# Autodesk Inventor assembly: Leg_joint_roll_pitch
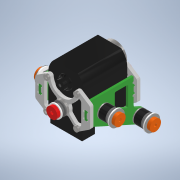
[picture p0: Inventor's stored thumbnail of the model, 180x180]
Saved by Autodesk Inventor 2020.4 (Build 244396000, 396)
## iProperties
Part Number: Leg_joint_roll_pitch
Document SubType Name: Assembly
Designer: Masato Kubotera
Mass: 101.309 g
Surface Area: 368.925 cm^2
Volume: 74.117 cm^3
Density: 1.36688 g/cm^3
Author: Masato Kubotera
## Documents named in this file (22)
- C:\Users\Masato\Documents\Inventor\CIT Brains_Inventor\SUSTAINA-OP\LowerBody\Leg_joit\Leg_joint_roll_pitch.iam
- C:\Users\Masato\Documents\Inventor\CIT Brains_Inventor\SUSTAINA-OP\LowerBody\Leg_joit\Leg_joint_pitch_frame.ipt
- C:\Users\Masato\Documents\Inventor\CIT Brains_Inventor\SUSTAINA-OP\LowerBody\Leg_joit\Leg_joint_roll_frame.ipt
- C:\Users\Masato\Documents\Inventor\CIT Brains_Inventor\SUSTAINA-OP\ReadyMade\KONDO\B3M-SC-1170-A.ipt
- C:\Users\Masato\Documents\Inventor\CIT Brains_Inventor\SUSTAINA-OP\ReadyMade\Screw\M2_6-20.ipt
- C:\Users\Masato\Documents\Inventor\CIT Brains_Inventor\SUSTAINA-OP\ReadyMade\Screw\M2_6-15.ipt
- C:\Users\Masato\Documents\Inventor\CIT Brains_Inventor\SUSTAINA-OP\ReadyMade\Bush\80F-0603.ipt
- C:\Users\Masato\Documents\Inventor\CIT Brains_Inventor\SUSTAINA-OP\ReadyMade\Washer\CC-0612-50B.ipt
- C:\Users\Masato\Documents\Inventor\CIT Brains_Inventor\SUSTAINA-OP\ReadyMade\InsertNut\SF419.ipt
- C:\Users\Masato\Documents\Inventor\CIT Brains_Inventor\SUSTAINA-OP\ReadyMade\Washer\UUW-0412-10H.ipt
- C:\Users\Masato\Documents\Inventor\CIT Brains_Inventor\SUSTAINA-OP\ReadyMade\Spacer\SLSBF6-39.5-M4-N4.ipt
- C:\Users\Masato\Documents\Inventor\CIT Brains_Inventor\SUSTAINA-OP\ReadyMade\Screw\DBTS4-11-6-DHC.ipt
- C:\Users\Masato\Documents\Inventor\CIT Brains_Inventor\SUSTAINA-OP\ReadyMade\Screw\DBTS4-5-5-DHC.ipt
- C:\Users\Masato\Documents\Inventor\CIT Brains_Inventor\SUSTAINA-OP\ReadyMade\Screw\DBTS4-10-4-DHC.ipt
- C:\Users\Masato\Documents\Inventor\CIT Brains_Inventor\SUSTAINA-OP\ReadyMade\InsertNut\S4-05-3W.ipt
- C:\Users\Masato\Documents\Inventor\CIT Brains_Inventor\SUSTAINA-OP\ReadyMade\KONDO\ClampHorn.ipt
- C:\Users\Masato\Documents\Inventor\CIT Brains_Inventor\SUSTAINA-OP\ReadyMade\Screw\620103008.ipt
- C:\Users\Masato\Documents\Inventor\CIT Brains_Inventor\SUSTAINA-OP\ReadyMade\Screw\DBTS4-11-8-DHC.ipt
- C:\Users\Masato\Documents\Inventor\CIT Brains_Inventor\SUSTAINA-OP\ReadyMade\Washer\UUW-0614-05H.ipt
- C:\Users\Masato\Documents\Inventor\CIT Brains_Inventor\SUSTAINA-OP\ReadyMade\Washer\TT-0612-10.ipt
- C:\Users\Masato\Documents\Inventor\CIT Brains_Inventor\SUSTAINA-OP\ReadyMade\Washer\TT-0814-10.ipt
- C:\Users\Masato\Documents\Inventor\CIT Brains_Inventor\SUSTAINA-OP\ReadyMade\Washer\CCC-0612-65B.ipt
## Components (52 placed, 21 different names)
1. B3M-SC-1170-A:1 — 挿入:1, 挿入:2, 挿入:3, 挿入:4, 挿入:11, 挿入:12, 挿入:13, 挿入:14, メイト:1, メイト:2, フラッシュ:1, 挿入:49, 角度:3, 挿入:50
2. Leg_joint_roll_frame:1 — 挿入:1, 挿入:2, 挿入:3, 挿入:4, 挿入:5, 挿入:6, 挿入:7, 挿入:8, 挿入:9, 挿入:10, 角度:1, フラッシュ:2, メイト:3, メイト:4, メイト:5
3. Leg_joint_roll_frame:2 — 挿入:11, 挿入:12, 挿入:13, 挿入:14, 挿入:15, 挿入:16, 挿入:17, 挿入:18, 角度:2, 角度:4
4. Leg_joint_pitch_frame:1 — フラッシュ:3, 挿入:19, フラッシュ:4, メイト:5, 挿入:20, 挿入:21, 挿入:22
5. Leg_joint_pitch_frame:2 — フラッシュ:2, フラッシュ:3, フラッシュ:4, メイト:3, メイト:4, 挿入:23, 挿入:24, 挿入:25, 挿入:26
6. 80F-0603:1 — 挿入:43
7. 80F-0603:2 — 挿入:44
8. 80F-0603:3 — 挿入:243
9. 80F-0603:4 — 挿入:242
10. 80F-0603:5 — 挿入:244
11. 80F-0603:6 — 挿入:245
12. UUW-0412-10BH:1 — 挿入:9, 挿入:27
13. UUW-0412-10BH:2 — 挿入:17, 挿入:28, 挿入:33
14. UUW-0412-10BH:3 — 挿入:19, 挿入:226, 挿入:241
15. UUW-0412-10BH:4 — 挿入:22, 挿入:35, 挿入:240
16. UUW-0412-10BH:5 — 挿入:23, 挿入:227, 挿入:239
17. UUW-0412-10BH:6 — 挿入:26, 挿入:37, 挿入:238
18. UUW-0412-10BH:7 — 挿入:27, 挿入:38, 挿入:43
19. CC-0612-50B:5 — 挿入:28, 挿入:44
20. SF419:1 — 挿入:25
21. SF419:2 — 挿入:20
22. S4-05-3W:1 — 挿入:10, 角度:1
23. S4-05-3W:2 — 挿入:18, 角度:2
24. SLSBF6-39.5-M4-N4:1 — 挿入:21, 挿入:24, 角度:4
25. DBS4-5-5:1 — 挿入:38, 挿入:232
26. DBTS4-11-6:3 — 挿入:37, 挿入:229
27. DBTS4-11-6:4 — 挿入:35, 挿入:230
28. DBTS4-10-4:1 — 挿入:33, 挿入:233
29. ClampHorn:1 — 挿入:49, 角度:3
30. 620103008:1 — 挿入:50
31. DBTS4-11-8:1 — 挿入:226, 挿入:231
32. DBTS4-11-8:2 — 挿入:227, 挿入:228
33. UUW-0614-05BH:1 — 挿入:228, 挿入:234
34. UUW-0614-05BH:2 — 挿入:229, 挿入:235
35. UUW-0614-05BH:3 — 挿入:230, 挿入:236
36. UUW-0614-05BH:4 — 挿入:231, 挿入:237
37. TT-0612-10:1 — 挿入:233
38. TT-0612-10:2 — 挿入:232
39. TT-0814-10:1 — 挿入:234
40. TT-0814-10:2 — 挿入:235
41. TT-0814-10:3 — 挿入:237
42. TT-0814-10:4 — 挿入:236
43. CCC-0612-65B:1 — 挿入:238, 挿入:245
44. CCC-0612-65B:2 — 挿入:241, 挿入:243
45. CCC-0612-65B:3 — 挿入:239, 挿入:244
46. CCC-0612-65B:4 — 挿入:240, 挿入:242
47. M2_6-20:1 — 挿入:7
48. M2_6-20:2 — 挿入:8
49. M2_6-20:3 — 挿入:5
50. M2_6-20:4 — 挿入:6
51. M2_6-15:2 — 挿入:16
52. M2_6-15:3 — 挿入:15
## Relationships (69: Insert 56, Mate 5, Flush 4, Angle 4)
- フラッシュ:1 [Flush]: B3M-SC-1170-A:1
- メイト:1 [Mate]: B3M-SC-1170-A:1
- メイト:2 [Mate]: B3M-SC-1170-A:1
- 挿入:1 [Insert]: B3M-SC-1170-A:1 ↔ Leg_joint_roll_frame:1
- 挿入:2 [Insert]: B3M-SC-1170-A:1 ↔ Leg_joint_roll_frame:1
- 挿入:3 [Insert]: B3M-SC-1170-A:1 ↔ Leg_joint_roll_frame:1
- 挿入:4 [Insert]: B3M-SC-1170-A:1 ↔ Leg_joint_roll_frame:1
- 挿入:5 [Insert]: Leg_joint_roll_frame:1 ↔ M2_6-20:3
- 挿入:6 [Insert]: Leg_joint_roll_frame:1 ↔ M2_6-20:4
- 挿入:7 [Insert]: Leg_joint_roll_frame:1 ↔ M2_6-20:1
- 挿入:8 [Insert]: Leg_joint_roll_frame:1 ↔ M2_6-20:2
- 挿入:9 [Insert]: Leg_joint_roll_frame:1 ↔ UUW-0412-10BH:1
- 挿入:10 [Insert]: Leg_joint_roll_frame:1 ↔ S4-05-3W:1
- 角度:1 [Angle] (0 deg): Leg_joint_roll_frame:1 ↔ S4-05-3W:1
- 挿入:11 [Insert]: B3M-SC-1170-A:1 ↔ Leg_joint_roll_frame:2
- 挿入:12 [Insert]: B3M-SC-1170-A:1 ↔ Leg_joint_roll_frame:2
- 挿入:13 [Insert]: B3M-SC-1170-A:1 ↔ Leg_joint_roll_frame:2
- 挿入:14 [Insert]: B3M-SC-1170-A:1 ↔ Leg_joint_roll_frame:2
- 挿入:15 [Insert]: Leg_joint_roll_frame:2 ↔ M2_6-15:3
- 挿入:16 [Insert]: Leg_joint_roll_frame:2 ↔ M2_6-15:2
- 挿入:17 [Insert]: Leg_joint_roll_frame:2 ↔ UUW-0412-10BH:2
- 挿入:18 [Insert]: Leg_joint_roll_frame:2 ↔ S4-05-3W:2
- 角度:2 [Angle] (0 deg): Leg_joint_roll_frame:2 ↔ S4-05-3W:2
- 挿入:19 [Insert]: Leg_joint_pitch_frame:1 ↔ UUW-0412-10BH:3
- 挿入:20 [Insert]: Leg_joint_pitch_frame:1 ↔ SF419:2
- 挿入:21 [Insert]: Leg_joint_pitch_frame:1 ↔ SLSBF6-39.5-M4-N4:1
- 挿入:22 [Insert]: Leg_joint_pitch_frame:1 ↔ UUW-0412-10BH:4
- 挿入:23 [Insert]: Leg_joint_pitch_frame:2 ↔ UUW-0412-10BH:5
- 挿入:24 [Insert]: Leg_joint_pitch_frame:2 ↔ SLSBF6-39.5-M4-N4:1
- 挿入:25 [Insert]: Leg_joint_pitch_frame:2 ↔ SF419:1
- 挿入:26 [Insert]: Leg_joint_pitch_frame:2 ↔ UUW-0412-10BH:6
- 挿入:27 [Insert]: UUW-0412-10BH:1 ↔ UUW-0412-10BH:7
- 挿入:28 [Insert]: UUW-0412-10BH:2 ↔ CC-0612-50B:5
- 挿入:33 [Insert]: UUW-0412-10BH:2 ↔ DBTS4-10-4:1
- 挿入:35 [Insert]: UUW-0412-10BH:4 ↔ DBTS4-11-6:4
- 挿入:37 [Insert]: UUW-0412-10BH:6 ↔ DBTS4-11-6:3
- 挿入:38 [Insert]: UUW-0412-10BH:7 ↔ DBS4-5-5:1
- 挿入:43 [Insert]: 80F-0603:1 ↔ UUW-0412-10BH:7
- 挿入:44 [Insert]: 80F-0603:2 ↔ CC-0612-50B:5
- フラッシュ:2 [Flush]: Leg_joint_roll_frame:1 ↔ Leg_joint_pitch_frame:2
- フラッシュ:3 [Flush]: Leg_joint_pitch_frame:1 ↔ Leg_joint_pitch_frame:2
- フラッシュ:4 [Flush]: Leg_joint_pitch_frame:1 ↔ Leg_joint_pitch_frame:2
- メイト:3 [Mate] (0.025 mm): Leg_joint_roll_frame:1 ↔ Leg_joint_pitch_frame:2
- メイト:4 [Mate] (0.025 mm): Leg_joint_roll_frame:1 ↔ Leg_joint_pitch_frame:2
- メイト:5 [Mate] (0.025 mm): Leg_joint_roll_frame:1 ↔ Leg_joint_pitch_frame:1
- 挿入:49 [Insert]: B3M-SC-1170-A:1 ↔ ClampHorn:1
- 挿入:50 [Insert]: B3M-SC-1170-A:1 ↔ 620103008:1
- 角度:3 [Angle] (0 deg): B3M-SC-1170-A:1 ↔ ClampHorn:1
- 角度:4 [Angle] (0 deg): Leg_joint_roll_frame:2 ↔ SLSBF6-39.5-M4-N4:1
- 挿入:226 [Insert]: UUW-0412-10BH:3 ↔ DBTS4-11-8:1
- 挿入:227 [Insert]: UUW-0412-10BH:5 ↔ DBTS4-11-8:2
- 挿入:228 [Insert]: DBTS4-11-8:2 ↔ UUW-0614-05BH:1
- 挿入:229 [Insert]: DBTS4-11-6:3 ↔ UUW-0614-05BH:2
- 挿入:230 [Insert]: DBTS4-11-6:4 ↔ UUW-0614-05BH:3
- 挿入:231 [Insert]: DBTS4-11-8:1 ↔ UUW-0614-05BH:4
- 挿入:232 [Insert]: DBS4-5-5:1 ↔ TT-0612-10:2
- 挿入:233 [Insert]: DBTS4-10-4:1 ↔ TT-0612-10:1
- 挿入:234 [Insert]: UUW-0614-05BH:1 ↔ TT-0814-10:1
- 挿入:235 [Insert]: UUW-0614-05BH:2 ↔ TT-0814-10:2
- 挿入:236 [Insert]: UUW-0614-05BH:3 ↔ TT-0814-10:4
- 挿入:237 [Insert]: UUW-0614-05BH:4 ↔ TT-0814-10:3
- 挿入:238 [Insert]: UUW-0412-10BH:6 ↔ CCC-0612-65B:1
- 挿入:239 [Insert]: UUW-0412-10BH:5 ↔ CCC-0612-65B:3
- 挿入:240 [Insert]: UUW-0412-10BH:4 ↔ CCC-0612-65B:4
- 挿入:241 [Insert]: UUW-0412-10BH:3 ↔ CCC-0612-65B:2
- 挿入:242 [Insert]: 80F-0603:4 ↔ CCC-0612-65B:4
- 挿入:243 [Insert]: 80F-0603:3 ↔ CCC-0612-65B:2
- 挿入:244 [Insert]: 80F-0603:5 ↔ CCC-0612-65B:3
- 挿入:245 [Insert]: 80F-0603:6 ↔ CCC-0612-65B:1
